# Autodesk Inventor assembly: 2014 Recycle Rush Robot 1
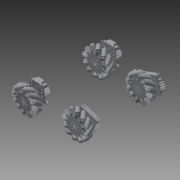
[picture p0: Inventor's stored thumbnail of the model, 180x180]
Saved by Autodesk Inventor 2014 (Build 180170000, 170)
## iProperties
Created: 2015-01-09
Part Number: 2014 Recycle Rush Robot 1
Document SubType Name: Assembly
Designer: student
Author: student
## Documents named in this file (5)
- C:\Users\student\Documents\Inventor\2015 Recycle Rush\2014 Recycle Rush Robot 1.iam
- C:\Users\student\Documents\Inventor\Dillon And Justin\Imported Components\am-0077a-500 Key Hub r2\am-0077a-500 Key Hub r2.ipt
- C:\Users\student\Documents\Inventor\Dillon And Justin\Imported Components\Toughbox mini (am-0654)\Toughbox mini (am-0654).iam
- C:\Users\student\Documents\Inventor\Dillon And Justin\Imported Components\8 inch mecanum left wheel\8 inch mecanum left wheel.iam
- C:\Users\student\Documents\Inventor\Dillon And Justin\Imported Components\8 inch mecanum right wheel\8 inch mecanum right wheel.iam
## Components (12 placed, 4 different names)
1. am-0077a-500 Key Hub r2:1 — Mate:4, Mate:5, Mate:6, Mate:7, Mate:8
2. Toughbox mini (am-0654):1 [sub-assembly] — Mate:4, Mate:5
3. 8 inch mecanum left wheel:1 [sub-assembly] — Mate:6, Mate:7, Mate:8
4. 8 inch mecanum right wheel:1 [sub-assembly] — Mate:9, Mate:10, Mate:16
5. am-0077a-500 Key Hub r2:2 — Mate:9, Mate:10, Mate:11, Mate:12, Mate:16
6. Toughbox mini (am-0654):2 [sub-assembly] — Mate:11, Mate:12
7. 8 inch mecanum left wheel:2 [sub-assembly] — Mate:13, Mate:14
8. am-0077a-500 Key Hub r2:3 — Mate:13, Mate:14, Mate:15
9. Toughbox mini (am-0654):3 [sub-assembly] — Mate:15
10. 8 inch mecanum right wheel:2 [sub-assembly] — Mate:17, Mate:18, Mate:19
11. am-0077a-500 Key Hub r2:4 — Mate:17, Mate:18, Mate:19, Mate:20
12. Toughbox mini (am-0654):4 [sub-assembly] — Mate:20
## Relationships (17: Mate 17)
- Mate:4: am-0077a-500 Key Hub r2:1 ↔ Toughbox mini (am-0654):1
- Mate:5: am-0077a-500 Key Hub r2:1 ↔ Toughbox mini (am-0654):1
- Mate:6: am-0077a-500 Key Hub r2:1 ↔ 8 inch mecanum left wheel:1
- Mate:7: am-0077a-500 Key Hub r2:1 ↔ 8 inch mecanum left wheel:1
- Mate:8: am-0077a-500 Key Hub r2:1 ↔ 8 inch mecanum left wheel:1
- Mate:9: 8 inch mecanum right wheel:1 ↔ am-0077a-500 Key Hub r2:2
- Mate:10: 8 inch mecanum right wheel:1 ↔ am-0077a-500 Key Hub r2:2
- Mate:11: am-0077a-500 Key Hub r2:2 ↔ Toughbox mini (am-0654):2
- Mate:12: am-0077a-500 Key Hub r2:2 ↔ Toughbox mini (am-0654):2
- Mate:13: 8 inch mecanum left wheel:2 ↔ am-0077a-500 Key Hub r2:3
- Mate:14: 8 inch mecanum left wheel:2 ↔ am-0077a-500 Key Hub r2:3
- Mate:15: am-0077a-500 Key Hub r2:3 ↔ Toughbox mini (am-0654):3
- Mate:16: 8 inch mecanum right wheel:1 ↔ am-0077a-500 Key Hub r2:2
- Mate:17: 8 inch mecanum right wheel:2 ↔ am-0077a-500 Key Hub r2:4
- Mate:18: 8 inch mecanum right wheel:2 ↔ am-0077a-500 Key Hub r2:4
- Mate:19: 8 inch mecanum right wheel:2 ↔ am-0077a-500 Key Hub r2:4
- Mate:20: am-0077a-500 Key Hub r2:4 ↔ Toughbox mini (am-0654):4
